# Autodesk Inventor assembly: spur_gear_m0.8-18.4
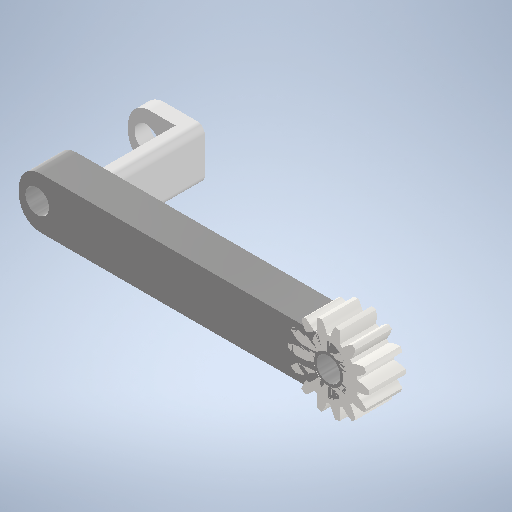
[picture p0: Inventor's stored thumbnail of the model, 512x512]
Saved by Autodesk Inventor 2025 (Build 290162000, 162)
## iProperties
Created: 2025-09-11
Part Number: spur_gear_m0.8-18.4
Document SubType Name: Assembly
Designer: sooo1
Author: sooo1
## Documents named in this file (4)
- C:\Users\sooo1\Downloads\final-20260216T060151Z-1-001\final\stroke_module\link_arm2_p1.iam
- C:\Users\sooo1\Downloads\final-20260216T060151Z-1-001\final\stroke_module\link_arm1_2.iam
- C:\Users\sooo1\Downloads\final-20260216T060151Z-1-001\final\stroke_module\平歯車1.iam
- C:\Users\sooo1\Downloads\final-20260216T060151Z-1-001\final\stroke_module\guide_link_2.ipt
## Components (3 placed, 3 different names)
1. link_arm1_2:1 [sub-assembly] — メイト:1, フラッシュ:8, メイト:3, メイト:7, フラッシュ:11, 角度:1, メイト:10, メイト:11, フラッシュ:12
2. 平歯車:1 [sub-assembly] — メイト:7, フラッシュ:11, 角度:1
3. guide_link_2:1 — メイト:10, メイト:11, フラッシュ:12
## Relationships (9: Mate 5, Flush 3, Angle 1)
- メイト:1 [Mate]: link_arm1_2:1
- フラッシュ:8 [Flush]: link_arm1_2:1
- メイト:3 [Mate]: link_arm1_2:1
- メイト:7 [Mate]: link_arm1_2:1 ↔ 平歯車:1
- フラッシュ:11 [Flush]: link_arm1_2:1 ↔ 平歯車:1
- 角度:1 [Angle] (90 deg): link_arm1_2:1 ↔ 平歯車:1
- メイト:10 [Mate]: link_arm1_2:1 ↔ guide_link_2:1
- メイト:11 [Mate]: link_arm1_2:1 ↔ guide_link_2:1
- フラッシュ:12 [Flush]: link_arm1_2:1 ↔ guide_link_2:1
